# Autodesk Inventor assembly: DrumCam
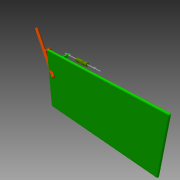
[picture p0: Inventor's stored thumbnail of the model, 180x180]
Saved by Autodesk Inventor 2015 (Build 190159000, 159)
## iProperties
Created: 2015-04-28
Part Number: DrumCam
Document SubType Name: Assembly
Designer: WASHHSST
Author: WASHHSST
## Documents named in this file (4)
- C:\Users\washhsst\Documents\GitHub\myWork\DrumCam\DrumCam.iam
- C:\Users\washhsst\Documents\GitHub\myWork\DrumCam\BasePlate.ipt
- C:\Users\washhsst\Documents\GitHub\myWork\DrumCam\DrumCam.ipt
- C:\Users\washhsst\Documents\GitHub\myWork\DrumCam\SquareTubeSlider.ipt
## Components (3 placed, 3 different names)
1. BasePlate:1 — Mate:1, Mate:2
2. DrumCam:1 — Mate:1, Mate:2, Mate:3
3. SquareTubeSlider:1 — Mate:3
## Relationships (3: Mate 3)
- Mate:1: BasePlate:1 ↔ DrumCam:1
- Mate:2: BasePlate:1 ↔ DrumCam:1
- Mate:3: DrumCam:1 ↔ SquareTubeSlider:1
